# Autodesk Inventor assembly: assembly
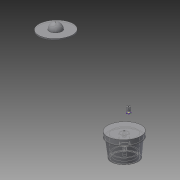
[picture p0: Inventor's stored thumbnail of the model, 180x180]
Saved by Autodesk Inventor 2014 (Build 180170000, 170)
## iProperties
Created: 2014-04-02
Part Number: assembly
Document SubType Name: Assembly
Designer: jferner
Author: jferner
## Documents named in this file (5)
- C:\Users\jferner\Downloads\flower\assembly.iam
- C:\Users\jferner\Downloads\flower\flower.ipt
- C:\Users\jferner\Downloads\flower\stem.ipt
- C:\Users\jferner\Downloads\flower\pot.ipt
- C:\Users\jferner\Downloads\flower\pot_bottom.ipt
## Components (4 placed, 4 different names)
1. flower:1
2. stem:1
3. pot:1 — Mate:1
4. pot_bottom:1 — Mate:1
## Relationships (1: Mate 1)
- Mate:1: pot:1 ↔ pot_bottom:1
